# Autodesk Inventor assembly: Electronics
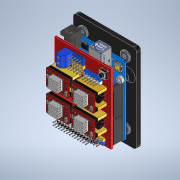
[picture p0: Inventor's stored thumbnail of the model, 180x180]
Saved by Autodesk Inventor 2022 (Build 260153000, 153)
## iProperties
Created: 2022-03-15
Part Number: Electronics
Document SubType Name: Assembly
Designer: JK
Author: JK
## Documents named in this file (7)
- C:\Users\JK\Documents\Inventor\ScaraNema\SCARA-3DP\Parts\Electronics\Electronics.iam
- C:\Users\JK\Documents\Inventor\ScaraNema\SCARA-3DP\Parts\Electronics\Electronics base.ipt
- C:\Users\JK\Documents\Inventor\ScaraNema\SCARA-3DP\Parts\Electronics\Arduino UNO and Shield\Arduino_CNC_Assembly.iam
- C:\Users\JK\Documents\Inventor\ScaraNema\SCARA-3DP\Parts\Fasteners\M3x10 socket bolt.ipt
- C:\Users\JK\Documents\Inventor\ScaraNema\SCARA-3DP\Parts\Fasteners\M3 Hex nut.ipt
- C:\Users\JK\Documents\Inventor\ScaraNema\SCARA-3DP\Parts\Fasteners\M5x8 Flat head bolt.ipt
- C:\Users\JK\Documents\Inventor\ScaraNema\SCARA-3DP\Parts\Fasteners\M5 T-Nut Drop-in 20x20.ipt
## Components (16 placed, 6 different names)
1. Electronics base:1 — Nivelación:1, Nivelación:2, Coincidencia:1, Coincidencia:8, Coincidencia:9, Coincidencia:10, Coincidencia:11, Ángulo:4, Ángulo:5, Coincidencia:16, Ángulo:8, Coincidencia:20
2. Arduino_CNC_Assembly:1 [sub-assembly] — Nivelación:1, Nivelación:2, Coincidencia:1, Coincidencia:2, Coincidencia:3, Coincidencia:4, Coincidencia:5, Coincidencia:6, Coincidencia:7
3. M3x10 socket bolt:1 — Coincidencia:4, Nivelación:4, Coincidencia:12
4. M3x10 socket bolt:2 — Coincidencia:3, Coincidencia:7, Nivelación:3, Coincidencia:14
5. M3x10 socket bolt:3 — Coincidencia:5, Coincidencia:6, Coincidencia:13
6. M3x10 socket bolt:4 — Coincidencia:2, Nivelación:3, Nivelación:4, Coincidencia:15
7. M5x8 Flat head bolt:1 — Coincidencia:8, Nivelación:6, Coincidencia:11, Coincidencia:19
8. M5x8 Flat head bolt:2 — Coincidencia:10, Nivelación:5, Coincidencia:17
9. M5x8 Flat head bolt:3 — Coincidencia:9, Nivelación:5, Nivelación:6, Coincidencia:18
10. M3 Hex nut:1 — Coincidencia:13, Nivelación:7, Nivelación:9, Ángulo:1, Ángulo:2, Ángulo:5
11. M3 Hex nut:2 — Coincidencia:12, Nivelación:9, Ángulo:1
12. M3 Hex nut:3 — Coincidencia:14, Nivelación:8, Ángulo:3, Ángulo:4
13. M3 Hex nut:4 — Coincidencia:15, Nivelación:7, Nivelación:8, Ángulo:2, Ángulo:3, Coincidencia:16
14. M5 T-Nut Drop-in 20x20:1 — Coincidencia:17, Ángulo:6, Nivelación:10
15. M5 T-Nut Drop-in 20x20:2 — Coincidencia:18, Ángulo:6, Ángulo:7, Nivelación:10, Nivelación:11
16. M5 T-Nut Drop-in 20x20:3 — Coincidencia:19, Ángulo:7, Ángulo:8, Nivelación:11, Coincidencia:20
## Relationships (39: Mate 20, Flush 11, Angle 8)
- Nivelación:1 [Flush] (5 mm): Electronics base:1 ↔ Arduino_CNC_Assembly:1
- Nivelación:2 [Flush] (5 mm): Electronics base:1 ↔ Arduino_CNC_Assembly:1
- Coincidencia:1 [Mate]: Electronics base:1 ↔ Arduino_CNC_Assembly:1
- Coincidencia:2 [Mate]: Arduino_CNC_Assembly:1 ↔ M3x10 socket bolt:4
- Coincidencia:3 [Mate]: Arduino_CNC_Assembly:1 ↔ M3x10 socket bolt:2
- Coincidencia:4 [Mate]: Arduino_CNC_Assembly:1 ↔ M3x10 socket bolt:1
- Coincidencia:5 [Mate]: Arduino_CNC_Assembly:1 ↔ M3x10 socket bolt:3
- Coincidencia:6 [Mate]: Arduino_CNC_Assembly:1 ↔ M3x10 socket bolt:3
- Coincidencia:7 [Mate]: Arduino_CNC_Assembly:1 ↔ M3x10 socket bolt:2
- Nivelación:3 [Flush]: M3x10 socket bolt:2 ↔ M3x10 socket bolt:4
- Nivelación:4 [Flush]: M3x10 socket bolt:1 ↔ M3x10 socket bolt:4
- Coincidencia:8 [Mate]: Electronics base:1 ↔ M5x8 Flat head bolt:1
- Coincidencia:9 [Mate]: Electronics base:1 ↔ M5x8 Flat head bolt:3
- Coincidencia:10 [Mate]: Electronics base:1 ↔ M5x8 Flat head bolt:2
- Nivelación:5 [Flush]: M5x8 Flat head bolt:2 ↔ M5x8 Flat head bolt:3
- Nivelación:6 [Flush]: M5x8 Flat head bolt:1 ↔ M5x8 Flat head bolt:3
- Coincidencia:11 [Mate]: Electronics base:1 ↔ M5x8 Flat head bolt:1
- Coincidencia:12 [Mate]: M3x10 socket bolt:1 ↔ M3 Hex nut:2
- Coincidencia:13 [Mate]: M3x10 socket bolt:3 ↔ M3 Hex nut:1
- Coincidencia:14 [Mate]: M3x10 socket bolt:2 ↔ M3 Hex nut:3
- Coincidencia:15 [Mate]: M3x10 socket bolt:4 ↔ M3 Hex nut:4
- Nivelación:7 [Flush]: M3 Hex nut:1 ↔ M3 Hex nut:4
- Nivelación:8 [Flush]: M3 Hex nut:3 ↔ M3 Hex nut:4
- Nivelación:9 [Flush]: M3 Hex nut:1 ↔ M3 Hex nut:2
- Ángulo:1 [Angle] (0 deg): M3 Hex nut:1 ↔ M3 Hex nut:2
- Ángulo:2 [Angle] (0 deg): M3 Hex nut:1 ↔ M3 Hex nut:4
- Ángulo:3 [Angle] (0 deg): M3 Hex nut:3 ↔ M3 Hex nut:4
- Ángulo:4 [Angle] (0 deg): Electronics base:1 ↔ M3 Hex nut:3
- Ángulo:5 [Angle] (0 deg): Electronics base:1 ↔ M3 Hex nut:1
- Coincidencia:16 [Mate]: Electronics base:1 ↔ M3 Hex nut:4
- Coincidencia:17 [Mate]: M5x8 Flat head bolt:2 ↔ M5 T-Nut Drop-in 20x20:1
- Coincidencia:18 [Mate]: M5x8 Flat head bolt:3 ↔ M5 T-Nut Drop-in 20x20:2
- Coincidencia:19 [Mate]: M5x8 Flat head bolt:1 ↔ M5 T-Nut Drop-in 20x20:3
- Ángulo:6 [Angle] (0 deg): M5 T-Nut Drop-in 20x20:1 ↔ M5 T-Nut Drop-in 20x20:2
- Ángulo:7 [Angle] (0 deg): M5 T-Nut Drop-in 20x20:2 ↔ M5 T-Nut Drop-in 20x20:3
- Ángulo:8 [Angle] (0 deg): Electronics base:1 ↔ M5 T-Nut Drop-in 20x20:3
- Nivelación:10 [Flush]: M5 T-Nut Drop-in 20x20:1 ↔ M5 T-Nut Drop-in 20x20:2
- Nivelación:11 [Flush]: M5 T-Nut Drop-in 20x20:2 ↔ M5 T-Nut Drop-in 20x20:3
- Coincidencia:20 [Mate] (0.6 mm): Electronics base:1 ↔ M5 T-Nut Drop-in 20x20:3
